# Autodesk Inventor assembly: LaundryRobot_v01
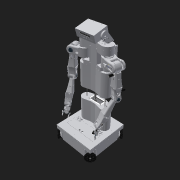
[picture p0: Inventor's stored thumbnail of the model, 180x180]
Saved by Autodesk Inventor 2017 SP1 (Build 210196100, 196)
## iProperties
Created: 2017-03-11
Part Number: LaundryRobot_v01
Document SubType Name: Assembly
Designer: zallen
Author: zallen
## Documents named in this file (4)
- C:\Users\Zach\Documents\GitHub\tr1\SlateTR1.iam
- C:\Users\Zach\Documents\GitHub\tr1\src\Body\Body.iam
- C:\Users\Zach\Documents\GitHub\tr1\src\Head\Head.iam
- C:\Users\Zach\Documents\GitHub\tr1\src\Base\Base.iam
## Components (3 placed, 3 different names)
1. Body:1 [sub-assembly] — Mate:31, Mate:42, Mate:37, Mate:38, Mate:41, Mate:43, Mate:44
2. Head:1 [sub-assembly] — Mate:41, Mate:43, Mate:44
3. Base:1 [sub-assembly] — Mate:11, Mate:12, Mate:23, Mate:31, Mate:42, Mate:37, Mate:38
## Relationships (10: Mate 10)
- Mate:11: Base:1
- Mate:12: Base:1
- Mate:23: Base:1
- Mate:31: Body:1 ↔ Base:1
- Mate:42: Body:1 ↔ Base:1
- Mate:37: Body:1 ↔ Base:1
- Mate:38: Body:1 ↔ Base:1
- Mate:41: Body:1 ↔ Head:1
- Mate:43: Body:1 ↔ Head:1
- Mate:44: Body:1 ↔ Head:1
